# Autodesk Inventor assembly: Matchboxscope_VCM_v1
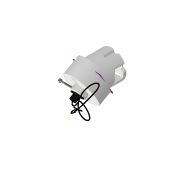
[picture p0: Inventor's stored thumbnail of the model, 180x180]
Saved by Autodesk Inventor 2022 (Build 260153000, 153)
## iProperties
Created: 2022-04-02
Part Number: Matchboxscope_VCM_v1
Document SubType Name: Assembly
Designer: Prakash Lab
Author: Prakash Lab
## Documents named in this file (11)
- C:\Users\diederichbenedict\Dropbox\Dokumente\Promotion\PROJECTS\Matchboxscope\INVENTOR\MATCHBOXSCOPE\Spectroscope_v0.iam
- C:\Users\diederichbenedict\Dropbox\Dokumente\Promotion\PROJECTS\Matchboxscope\INVENTOR\MATCHBOXSCOPE\Matchboxscope_bottom_v0.ipt
- C:\Users\diederichbenedict\Dropbox\Dokumente\Promotion\PROJECTS\Matchboxscope\INVENTOR\MATCHBOXSCOPE\00_ESP3-CAM.iam
- C:\Users\diederichbenedict\Dropbox\Dokumente\Promotion\PROJECTS\Matchboxscope\INVENTOR\MATCHBOXSCOPE\00_Powerbank.ipt
- C:\Users\diederichbenedict\Documents\Inventor\Content Center Files\R2022\de-DE\DIN 912\DIN 912 - M3 x 0.5 x 25 x 18.ipt
- C:\Users\diederichbenedict\Dropbox\Dokumente\Promotion\PROJECTS\Matchboxscope\INVENTOR\MATCHBOXSCOPE\Spectrometer_gratingholder_v0.ipt
- C:\Users\diederichbenedict\Dropbox\Dokumente\Promotion\PROJECTS\Matchboxscope\INVENTOR\MATCHBOXSCOPE\00_Grating_1000linesPerMM.ipt
- C:\Users\diederichbenedict\Dropbox\Dokumente\Promotion\PROJECTS\Matchboxscope\INVENTOR\MATCHBOXSCOPE\Spectrometer_pinholeholder_v0.ipt
- C:\Users\diederichbenedict\Dropbox\Dokumente\Promotion\PROJECTS\Matchboxscope\INVENTOR\MATCHBOXSCOPE\00_mk8_nozzle_0.4STEP.ipt
- C:\Users\diederichbenedict\Dropbox\Dokumente\Promotion\PROJECTS\Matchboxscope\INVENTOR\MATCHBOXSCOPE\00_toslink_launcher_v3.ipt
- C:\Users\diederichbenedict\Dropbox\Dokumente\Promotion\PROJECTS\Matchboxscope\INVENTOR\MATCHBOXSCOPE\00_Toslink.ipt
## Components (14 placed, 10 different names)
1. Matchboxscope_bottom_v0:1 — Mate:1, Mate:2, Mate:3, Mate:4, Flush:1, Fluchtend:2, Einfügen:1, Fluchtend:3, Passend:5, Fluchtend:4
2. 00_ESP3-CAM:1 [sub-assembly] — Mate:4, Flush:1, Fluchtend:2
3. 00_Powerbank:1
4. DIN 912 - ersetzt durch DIN EN ISO 4762 M3 x 25:4
5. DIN 912 - ersetzt durch DIN EN ISO 4762 M3 x 25:5
6. DIN 912 - ersetzt durch DIN EN ISO 4762 M3 x 25:6
7. DIN 912 - ersetzt durch DIN EN ISO 4762 M3 x 25:7
8. Spectrometer_gratingholder_v0:1 — Einfügen:1, Tangential:1, Fluchtend:4
9. 00_Grating_1000linesPerMM:1 — Fluchtend:3, Passend:5, Tangential:1, Fluchtend:5
10. Spectrometer_pinholeholder_v0:1 — Fluchtend:5, Einfügen:2
11. 00_mk8_nozzle_0.4STEP:1 — Einfügen:2, Einfügen:3
12. 00_toslink_launcher_v3:1 — Einfügen:3, Einfügen:4, Passend:6
13. 00_Toslink:1 — Einfügen:4
14. DIN 912 - ersetzt durch DIN EN ISO 4762 M3 x 25:8 — Passend:6
## Relationships (16: Mate 6, Flush 5, Insert 4, Tangent 1)
- Mate:1: Matchboxscope_bottom_v0:1
- Mate:2: Matchboxscope_bottom_v0:1
- Mate:3: Matchboxscope_bottom_v0:1
- Mate:4: Matchboxscope_bottom_v0:1 ↔ 00_ESP3-CAM:1
- Flush:1: Matchboxscope_bottom_v0:1 ↔ 00_ESP3-CAM:1
- Fluchtend:2 [Flush]: Matchboxscope_bottom_v0:1 ↔ 00_ESP3-CAM:1
- Einfügen:1 [Insert]: Matchboxscope_bottom_v0:1 ↔ Spectrometer_gratingholder_v0:1
- Fluchtend:3 [Flush]: Matchboxscope_bottom_v0:1 ↔ 00_Grating_1000linesPerMM:1
- Passend:5 [Mate] (2 mm): Matchboxscope_bottom_v0:1 ↔ 00_Grating_1000linesPerMM:1
- Tangential:1 (-2 mm): Spectrometer_gratingholder_v0:1 ↔ 00_Grating_1000linesPerMM:1
- Fluchtend:4 [Flush]: Matchboxscope_bottom_v0:1 ↔ Spectrometer_gratingholder_v0:1
- Fluchtend:5 [Flush]: 00_Grating_1000linesPerMM:1 ↔ Spectrometer_pinholeholder_v0:1
- Einfügen:2 [Insert]: Spectrometer_pinholeholder_v0:1 ↔ 00_mk8_nozzle_0.4STEP:1
- Einfügen:3 [Insert]: 00_mk8_nozzle_0.4STEP:1 ↔ 00_toslink_launcher_v3:1
- Einfügen:4 [Insert]: 00_toslink_launcher_v3:1 ↔ 00_Toslink:1
- Passend:6 [Mate]: 00_toslink_launcher_v3:1 ↔ DIN 912 - ersetzt durch DIN EN ISO 4762 M3 x 25:8
